# Autodesk Inventor assembly: Pancake Shifter Assembly
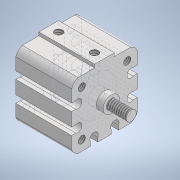
[picture p0: Inventor's stored thumbnail of the model, 180x180]
Saved by Autodesk Inventor 2021 (Build 250183000, 183)
## iProperties
Created: 2021-02-24
Part Number: Pancake Shifter Assembly
Document SubType Name: Assembly
Designer: aidan
Author: aidan
## Documents named in this file (3)
- C:\Users\aidan\Desktop\T3 Robotics\CAD\Generic and Stock\Pancake Shifter Assembly.iam
- C:\Users\aidan\Desktop\T3 Robotics\CAD\Generic and Stock\Pancake Shifter.ipt
- C:\Users\aidan\Desktop\T3 Robotics\CAD\Generic and Stock\Pancake Shifter Shaft.ipt
## Components (2 placed, 2 different names)
1. Pancake Shifter:1 — Mate:1
2. Pancake Shifter Shaft:1 — Mate:1
## Relationships (1: Mate 1)
- Mate:1: Pancake Shifter:1 ↔ Pancake Shifter Shaft:1
